# Autodesk Inventor assembly: RobotSpine
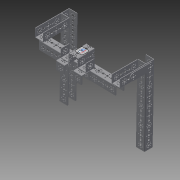
[picture p0: Inventor's stored thumbnail of the model, 180x180]
Saved by Autodesk Inventor 2015 (Build 190159000, 159)
## iProperties
Created: 2015-01-31
Part Number: RobotSpine
Document SubType Name: Assembly
Designer: sauhaarda
Author: sauhaarda
## Documents named in this file (9)
- C:\Users\sauhaarda\SkyDrive\Documents\Autodesk Workspace\RobotCad\RobotSpine.iam
- C:\Users\sauhaarda\SkyDrive\Documents\Autodesk Workspace\RobotCad\Imported Components\288mm Channel\Assembly3.iam
- C:\Users\sauhaarda\SkyDrive\Documents\Autodesk Workspace\RobotCad\Imported Components\Flat Bracket\Assembly4.iam
- C:\Users\sauhaarda\SkyDrive\Documents\Autodesk Workspace\RobotCad\Imported Components\96 mm Channel\Assembly5.iam
- C:\Users\sauhaarda\SkyDrive\Documents\Autodesk Workspace\RobotCad\Imported Components\288mm Channel\Assembly7.iam
- C:\Users\sauhaarda\SkyDrive\Documents\Autodesk Workspace\RobotCad\Imported Components\288mm Channel\Assembly8.iam
- C:\Users\sauhaarda\SkyDrive\Documents\Autodesk Workspace\RobotCad\Imported Components\32mm Channel\Assembly10.iam
- C:\Users\sauhaarda\SkyDrive\Documents\Autodesk Workspace\RobotCad\Imported Components\32mm Channel\Assembly19.iam
- C:\Users\sauhaarda\SkyDrive\Documents\Autodesk Workspace\RobotCad\Imported Components\64 mm Channel\Assembly18.iam
## Components (12 placed, 8 different names)
1. Assembly3:2 [sub-assembly] — Insert:1, Angle:1
2. Assembly4:1 [sub-assembly] — Insert:1, Angle:1, Insert:2, Angle:2
3. Assembly5:1 [sub-assembly] — Insert:2, Angle:2, Angle:7, Insert:7
4. Assembly7:1 [sub-assembly] — Angle:4, Angle:7, Mate:1, Mate:2, Flush:1, Flush:2, Insert:6, Insert:7, Insert:8, Insert:9, Mate:3, Mate:4, Insert:10, Insert:13
5. Assembly5:2 [sub-assembly] — Insert:4, Angle:4, Angle:5, Insert:6
6. Assembly4:2 [sub-assembly] — Insert:4, Insert:5, Angle:3, Angle:5, Angle:6
7. Assembly8:1 [sub-assembly] — Insert:5, Angle:3, Angle:6
8. Assembly10:1 [sub-assembly] — Mate:1, Flush:2, Insert:9, Insert:12
9. Assembly10:2 [sub-assembly] — Mate:2, Flush:1, Insert:8, Insert:11
10. Assembly19:1 [sub-assembly] — Mate:3, Insert:10, Insert:11, Flush:4
11. Assembly19:2 [sub-assembly] — Mate:4, Insert:12, Insert:13, Flush:5
12. Assembly18:1 [sub-assembly] — Flush:4, Flush:5
## Relationships (27: Insert 12, Angle 7, Mate 4, Flush 4)
- Insert:1: Assembly3:2 ↔ Assembly4:1
- Angle:1 (0 deg): Assembly3:2 ↔ Assembly4:1
- Insert:2: Assembly4:1 ↔ Assembly5:1
- Angle:2 (0 deg): Assembly4:1 ↔ Assembly5:1
- Insert:4: Assembly5:2 ↔ Assembly4:2
- Insert:5: Assembly4:2 ↔ Assembly8:1
- Angle:3 (0 deg): Assembly4:2 ↔ Assembly8:1
- Angle:4 (0 deg): Assembly7:1 ↔ Assembly5:2
- Angle:5 (0 deg): Assembly5:2 ↔ Assembly4:2
- Angle:6 (0 deg): Assembly4:2 ↔ Assembly8:1
- Angle:7 (0 deg): Assembly5:1 ↔ Assembly7:1
- Mate:1: Assembly7:1 ↔ Assembly10:1
- Mate:2: Assembly7:1 ↔ Assembly10:2
- Flush:1: Assembly7:1 ↔ Assembly10:2
- Flush:2: Assembly7:1 ↔ Assembly10:1
- Insert:6: Assembly7:1 ↔ Assembly5:2
- Insert:7: Assembly5:1 ↔ Assembly7:1
- Insert:8: Assembly7:1 ↔ Assembly10:2
- Insert:9: Assembly7:1 ↔ Assembly10:1
- Mate:3: Assembly7:1 ↔ Assembly19:1
- Mate:4: Assembly7:1 ↔ Assembly19:2
- Insert:10: Assembly7:1 ↔ Assembly19:1
- Insert:11: Assembly10:2 ↔ Assembly19:1
- Insert:12: Assembly10:1 ↔ Assembly19:2
- Insert:13: Assembly7:1 ↔ Assembly19:2
- Flush:4: Assembly19:1 ↔ Assembly18:1
- Flush:5: Assembly19:2 ↔ Assembly18:1
